# Autodesk Inventor assembly: socket presentation
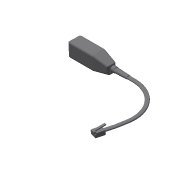
[picture p0: Inventor's stored thumbnail of the model, 180x180]
Saved by Autodesk Inventor 2022 Beta2 (Build 260130000, 130) ContinuousBuild 0
## iProperties
Created: 2007-04-03
Part Number: socket presentation
Document SubType Name: Assembly
Designer: PMILLER
Author: PMILLER
## Documents named in this file (6)
- C:\Autodesk Inventor 2021 Intro Practice Files\socket presentation.iam
- C:\Autodesk Inventor 2021 Intro Practice Files\encbase.ipt
- C:\Autodesk Inventor 2021 Intro Practice Files\pcb.ipt
- C:\Autodesk Inventor 2021 Intro Practice Files\connect.ipt
- C:\Autodesk Inventor 2021 Intro Practice Files\enctop.ipt
- C:\Autodesk Inventor 2021 Intro Practice Files\wire presentation.ipt
## Components (5 placed, 5 different names)
1. encbase:1 — Insert:1, Angle:1, Insert:3, Mate:1, Flush:1, Flush:2, Mate:2
2. pcb:1 — Insert:1, Angle:1, Insert:2
3. connect:1 — Insert:2
4. wire presentation:1 — Insert:3, Mate:1
5. enctop:1 — Flush:1, Flush:2, Mate:2
## Relationships (9: Insert 3, Angle 2, Mate 2, Flush 2)
- Insert:1 (-6.985 mm): encbase:1 ↔ pcb:1
- Angle:1 (180 deg): encbase:1 ↔ pcb:1
- [Angle] (180 deg): pcb:1 ↔ connect:1
- Insert:2: pcb:1 ↔ connect:1
- Insert:3: encbase:1 ↔ wire presentation:1
- Mate:1: encbase:1 ↔ wire presentation:1
- Flush:1: encbase:1 ↔ enctop:1
- Flush:2: encbase:1 ↔ enctop:1
- Mate:2: encbase:1 ↔ enctop:1
